# Autodesk Inventor assembly: 3361479 HGPL-14-20-A-B---(0)
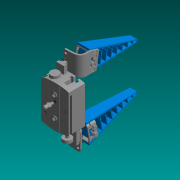
[picture p0: Inventor's stored thumbnail of the model, 180x180]
Saved by Autodesk Inventor 2020.3 (Build 243373000, 373)
## iProperties
Part Number: 3361479 HGPL-14-20-A-B---(0)
Catalog Web Link: www.cadenas.de
Description: HGPL-B-Parallel gripper
Vendor: FESTO
Document SubType Name: Assembly
Designer: partserver
Manufacturer: FESTO
Mass: 305 g
Surface Area: 358.431 cm^2
Volume: 79.5066 cm^3
Density: 3.83616 g/cm^3
Category: PARTsolutions
Company: FESTO
PSOL_IDENT_0: {ATYP=ASSISTANT},{DATA=script=$CADENAS_DATA/23d-libs/festo/webfesto.vbb/&M_FAMILY=HGPL&M_GROUP=01&M_
PSOL_IDENT_1: PARTNO=3361479&IDCODE1=HGPL-14-20-A-B&IDCODE2=&customer_number_cns=&MATES=1&LOD=HI&LOCKERP=0&SINGLEP
PSOL_IDENT_2: ART=1}
NB: 3361479 HGPL-14-20-A-B---(0)
NN: HGPL-B
NT: Parallel gripper
NBSYN: $TNR. $TYP.---($HUBST.)
LINA: 3361479 HGPL-14-20-A-B---(0)
CATALOG: Festo
TNR: 3361479
TYP: HGPL-14-20-A-B
KDM: 14
HUB: 20
HUBST: 0
L1: 73.6
L2: 36
L3: 0
L4: 62
L5: 22
L6: 8
H1: 30
H2: 29
H3: 24.4
H4: 10
H5: 12
H6: 11.2
H7: 0
H10: 4
B1: 48
B2: 34.5
B3: 22
B4: 40
G3: M3
T6: 6.5
CNSMASSEXACT: 0.305
SUPPLIER: FESTO
ARTICLENO: 3361479 HGPL-14-20-A-B---(0)
BOMINFO: 3361479 HGPL-14-20-A-B---(0)
CREATOR: CADENAS GmbH
Title: 3361479 HGPL-14-20-A-B---(0)
Author: Cadenas PARTsolutions
Comments: Parallel gripper
## Documents named in this file (9)
- C:\Users\Svend\OneDrive\Documents\GitHub\BeerMinder\3D-model\servo\AIS2020\3361479 HGPL-14-20-A-B---(0).iam
- C:\Users\Svend\OneDrive\Documents\GitHub\BeerMinder\3D-model\servo\AIS2020\3361628 HGPL-14-20-A-B---(GEH).ipt
- C:\Users\Svend\OneDrive\Documents\GitHub\BeerMinder\3D-model\servo\AIS2020\3361610 HGPL-BAC-14-20---(J).ipt
- C:\Users\Svend\OneDrive\Documents\GitHub\BeerMinder\3D-model\servo\AIS2020\189652 ZBH-5.ipt
- C:\Users\Svend\OneDrive\Documents\GitHub\BeerMinder\3D-model\servo\AIS2020\DIN-913 - M3x3.ipt
- C:\Users\Svend\OneDrive\Documents\GitHub\BeerMinder\3D-model\servo\AIS2020\DIN-913 - M5x5.ipt
- C:\Users\Svend\OneDrive\Documents\GitHub\BeerMinder\3D-model\servo\AIS2020\DIN-71412 A M5x0_8_SW7.ipt
- C:\Users\Svend\OneDrive\Documents\GitHub\BeerMinder\3D-model\servo\AIS2020\150927 ZBH-9.ipt
- C:\Users\Svend\OneDrive\Documents\GitHub\BeerMinder\3D-model\gripper\AGf.iam
## Components (16 placed, 8 different names)
1. 3361628 HGPL-14-20-A-B---(GEH):1 — JAW1_Z@1 <-> ANBAU_Z@2, JAW1_YZ@1 <-> ANBAU_YZ@2, PIN_1_XY@1 <-> IP1_XY@8, PIN_1_Z@1 <-> IP1_Z@8, PIN_1_YZ@1 <-> IP1_YZ@8, PIN_2_XY@1 <-> IP1_XY@9, PIN_2_Z@1 <-> IP1_Z@9, PIN_2_YZ@1 <-> IP1_YZ@9, NIPPEL_OBEN_XY@1 <-> IP1_XY@10, NIPPEL_OBEN_Z@1 <-> IP1_Z@10, NIPPEL_OBEN_YZ@1 <-> IP1_YZ@10, NIPPEL_UNTEN_XY@1 <-> IP1_XY@11, NIPPEL_UNTEN_Z@1 <-> IP1_Z@11, NIPPEL_UNTEN_YZ@1 <-> IP1_YZ@11, NIPPEL_XY@1 <-> ANBAU_XY@12, NIPPEL_Z@1 <-> ANBAU_Z@12, NIPPEL_YZ@1 <-> ANBAU_YZ@12, ZBH_UNTEN_1_XY@1 <-> insert_XY@13, ZBH_UNTEN_1_Z@1 <-> insert_Z@13, ZBH_UNTEN_1_YZ@1 <-> insert_YZ@13, ZBH_UNTEN_2_XY@1 <-> insert_XY@14, ZBH_UNTEN_2_Z@1 <-> insert_Z@14, ZBH_UNTEN_2_YZ@1 <-> insert_YZ@14, Mate:22, Mate:23
2. 3361610 HGPL-BAC-14-20---(J):1 — JAW1_Z@1 <-> ANBAU_Z@2, JAW1_YZ@1 <-> ANBAU_YZ@2, ZBHJAW1_XY@2 <-> insert_XY@3, ZBHJAW1_Z@2 <-> insert_Z@3, ZBHJAW1_YZ@2 <-> insert_YZ@3, ZBHJAW2_XY@2 <-> insert_XY@4, ZBHJAW2_Z@2 <-> insert_Z@4, ZBHJAW2_YZ@2 <-> insert_YZ@4, Mate:25, Angle:14, Mate:26
3. 189652 ZBH-5:1 — ZBHJAW1_XY@2 <-> insert_XY@3, ZBHJAW1_Z@2 <-> insert_Z@3, ZBHJAW1_YZ@2 <-> insert_YZ@3
4. 189652 ZBH-5:2 — ZBHJAW2_XY@2 <-> insert_XY@4, ZBHJAW2_Z@2 <-> insert_Z@4, ZBHJAW2_YZ@2 <-> insert_YZ@4
5. 3361610 HGPL-BAC-14-20---(J):2 — ZBHJAW1_XY@5 <-> insert_XY@6, ZBHJAW1_Z@5 <-> insert_Z@6, ZBHJAW1_YZ@5 <-> insert_YZ@6, ZBHJAW2_XY@5 <-> insert_XY@7, ZBHJAW2_Z@5 <-> insert_Z@7, ZBHJAW2_YZ@5 <-> insert_YZ@7, Mate:22, Mate:23, Mate:24, Angle:13, Mate:27
6. 189652 ZBH-5:3 — ZBHJAW1_XY@5 <-> insert_XY@6, ZBHJAW1_Z@5 <-> insert_Z@6, ZBHJAW1_YZ@5 <-> insert_YZ@6
7. 189652 ZBH-5:4 — ZBHJAW2_XY@5 <-> insert_XY@7, ZBHJAW2_Z@5 <-> insert_Z@7, ZBHJAW2_YZ@5 <-> insert_YZ@7
8. DIN-913 - M3x3:1 — PIN_1_XY@1 <-> IP1_XY@8, PIN_1_Z@1 <-> IP1_Z@8, PIN_1_YZ@1 <-> IP1_YZ@8
9. DIN-913 - M3x3:2 — PIN_2_XY@1 <-> IP1_XY@9, PIN_2_Z@1 <-> IP1_Z@9, PIN_2_YZ@1 <-> IP1_YZ@9
10. DIN-913 - M5x5:1 — NIPPEL_OBEN_XY@1 <-> IP1_XY@10, NIPPEL_OBEN_Z@1 <-> IP1_Z@10, NIPPEL_OBEN_YZ@1 <-> IP1_YZ@10
11. DIN-913 - M5x5:2 — NIPPEL_UNTEN_XY@1 <-> IP1_XY@11, NIPPEL_UNTEN_Z@1 <-> IP1_Z@11, NIPPEL_UNTEN_YZ@1 <-> IP1_YZ@11
12. DIN-71412 A M5x0_8_SW7:1 — NIPPEL_XY@1 <-> ANBAU_XY@12, NIPPEL_Z@1 <-> ANBAU_Z@12, NIPPEL_YZ@1 <-> ANBAU_YZ@12
13. 150927 ZBH-9:1 — ZBH_UNTEN_1_XY@1 <-> insert_XY@13, ZBH_UNTEN_1_Z@1 <-> insert_Z@13, ZBH_UNTEN_1_YZ@1 <-> insert_YZ@13
14. 150927 ZBH-9:2 — ZBH_UNTEN_2_XY@1 <-> insert_XY@14, ZBH_UNTEN_2_Z@1 <-> insert_Z@14, ZBH_UNTEN_2_YZ@1 <-> insert_YZ@14
15. AGf:1 [sub-assembly] — Mate:24, Angle:13, Mate:27
16. AGf:2 [sub-assembly] — Mate:25, Angle:14, Mate:26
## Relationships (43: Mate 27, Angle 14, Flush 2)
- JAW1_Z@1 <-> ANBAU_Z@2 [Mate]: 3361628 HGPL-14-20-A-B---(GEH):1 ↔ 3361610 HGPL-BAC-14-20---(J):1
- JAW1_YZ@1 <-> ANBAU_YZ@2 [Angle] (0 deg): 3361628 HGPL-14-20-A-B---(GEH):1 ↔ 3361610 HGPL-BAC-14-20---(J):1
- ZBHJAW1_XY@2 <-> insert_XY@3 [Mate]: 3361610 HGPL-BAC-14-20---(J):1 ↔ 189652 ZBH-5:1
- ZBHJAW1_Z@2 <-> insert_Z@3 [Mate]: 3361610 HGPL-BAC-14-20---(J):1 ↔ 189652 ZBH-5:1
- ZBHJAW1_YZ@2 <-> insert_YZ@3 [Angle] (0 deg): 3361610 HGPL-BAC-14-20---(J):1 ↔ 189652 ZBH-5:1
- ZBHJAW2_XY@2 <-> insert_XY@4 [Mate]: 3361610 HGPL-BAC-14-20---(J):1 ↔ 189652 ZBH-5:2
- ZBHJAW2_Z@2 <-> insert_Z@4 [Mate]: 3361610 HGPL-BAC-14-20---(J):1 ↔ 189652 ZBH-5:2
- ZBHJAW2_YZ@2 <-> insert_YZ@4 [Angle] (0 deg): 3361610 HGPL-BAC-14-20---(J):1 ↔ 189652 ZBH-5:2
- ZBHJAW1_XY@5 <-> insert_XY@6 [Mate]: 3361610 HGPL-BAC-14-20---(J):2 ↔ 189652 ZBH-5:3
- ZBHJAW1_Z@5 <-> insert_Z@6 [Mate]: 3361610 HGPL-BAC-14-20---(J):2 ↔ 189652 ZBH-5:3
- ZBHJAW1_YZ@5 <-> insert_YZ@6 [Angle] (0 deg): 3361610 HGPL-BAC-14-20---(J):2 ↔ 189652 ZBH-5:3
- ZBHJAW2_XY@5 <-> insert_XY@7 [Mate]: 3361610 HGPL-BAC-14-20---(J):2 ↔ 189652 ZBH-5:4
- ZBHJAW2_Z@5 <-> insert_Z@7 [Mate]: 3361610 HGPL-BAC-14-20---(J):2 ↔ 189652 ZBH-5:4
- ZBHJAW2_YZ@5 <-> insert_YZ@7 [Angle] (0 deg): 3361610 HGPL-BAC-14-20---(J):2 ↔ 189652 ZBH-5:4
- PIN_1_XY@1 <-> IP1_XY@8 [Mate]: 3361628 HGPL-14-20-A-B---(GEH):1 ↔ DIN-913 - M3x3:1
- PIN_1_Z@1 <-> IP1_Z@8 [Mate]: 3361628 HGPL-14-20-A-B---(GEH):1 ↔ DIN-913 - M3x3:1
- PIN_1_YZ@1 <-> IP1_YZ@8 [Angle] (0 deg): 3361628 HGPL-14-20-A-B---(GEH):1 ↔ DIN-913 - M3x3:1
- PIN_2_XY@1 <-> IP1_XY@9 [Mate]: 3361628 HGPL-14-20-A-B---(GEH):1 ↔ DIN-913 - M3x3:2
- PIN_2_Z@1 <-> IP1_Z@9 [Mate]: 3361628 HGPL-14-20-A-B---(GEH):1 ↔ DIN-913 - M3x3:2
- PIN_2_YZ@1 <-> IP1_YZ@9 [Angle] (0 deg): 3361628 HGPL-14-20-A-B---(GEH):1 ↔ DIN-913 - M3x3:2
- NIPPEL_OBEN_XY@1 <-> IP1_XY@10 [Flush]: 3361628 HGPL-14-20-A-B---(GEH):1 ↔ DIN-913 - M5x5:1
- NIPPEL_OBEN_Z@1 <-> IP1_Z@10 [Mate]: 3361628 HGPL-14-20-A-B---(GEH):1 ↔ DIN-913 - M5x5:1
- NIPPEL_OBEN_YZ@1 <-> IP1_YZ@10 [Angle] (0 deg): 3361628 HGPL-14-20-A-B---(GEH):1 ↔ DIN-913 - M5x5:1
- NIPPEL_UNTEN_XY@1 <-> IP1_XY@11 [Flush]: 3361628 HGPL-14-20-A-B---(GEH):1 ↔ DIN-913 - M5x5:2
- NIPPEL_UNTEN_Z@1 <-> IP1_Z@11 [Mate]: 3361628 HGPL-14-20-A-B---(GEH):1 ↔ DIN-913 - M5x5:2
- NIPPEL_UNTEN_YZ@1 <-> IP1_YZ@11 [Angle] (0 deg): 3361628 HGPL-14-20-A-B---(GEH):1 ↔ DIN-913 - M5x5:2
- NIPPEL_XY@1 <-> ANBAU_XY@12 [Mate]: 3361628 HGPL-14-20-A-B---(GEH):1 ↔ DIN-71412 A M5x0_8_SW7:1
- NIPPEL_Z@1 <-> ANBAU_Z@12 [Mate]: 3361628 HGPL-14-20-A-B---(GEH):1 ↔ DIN-71412 A M5x0_8_SW7:1
- NIPPEL_YZ@1 <-> ANBAU_YZ@12 [Angle] (0 deg): 3361628 HGPL-14-20-A-B---(GEH):1 ↔ DIN-71412 A M5x0_8_SW7:1
- ZBH_UNTEN_1_XY@1 <-> insert_XY@13 [Mate]: 3361628 HGPL-14-20-A-B---(GEH):1 ↔ 150927 ZBH-9:1
- ZBH_UNTEN_1_Z@1 <-> insert_Z@13 [Mate]: 3361628 HGPL-14-20-A-B---(GEH):1 ↔ 150927 ZBH-9:1
- ZBH_UNTEN_1_YZ@1 <-> insert_YZ@13 [Angle] (0 deg): 3361628 HGPL-14-20-A-B---(GEH):1 ↔ 150927 ZBH-9:1
- ZBH_UNTEN_2_XY@1 <-> insert_XY@14 [Mate]: 3361628 HGPL-14-20-A-B---(GEH):1 ↔ 150927 ZBH-9:2
- ZBH_UNTEN_2_Z@1 <-> insert_Z@14 [Mate]: 3361628 HGPL-14-20-A-B---(GEH):1 ↔ 150927 ZBH-9:2
- ZBH_UNTEN_2_YZ@1 <-> insert_YZ@14 [Angle] (0 deg): 3361628 HGPL-14-20-A-B---(GEH):1 ↔ 150927 ZBH-9:2
- Mate:22: 3361628 HGPL-14-20-A-B---(GEH):1 ↔ 3361610 HGPL-BAC-14-20---(J):2
- Mate:23: 3361628 HGPL-14-20-A-B---(GEH):1 ↔ 3361610 HGPL-BAC-14-20---(J):2
- Mate:24: 3361610 HGPL-BAC-14-20---(J):2 ↔ AGf:1
- Mate:25: 3361610 HGPL-BAC-14-20---(J):1 ↔ AGf:2
- Angle:13 (180 deg): 3361610 HGPL-BAC-14-20---(J):2 ↔ AGf:1
- Angle:14 (180 deg): 3361610 HGPL-BAC-14-20---(J):1 ↔ AGf:2
- Mate:26: 3361610 HGPL-BAC-14-20---(J):1 ↔ AGf:2
- Mate:27: 3361610 HGPL-BAC-14-20---(J):2 ↔ AGf:1
